# Autodesk Inventor assembly: DriveMotorAssem
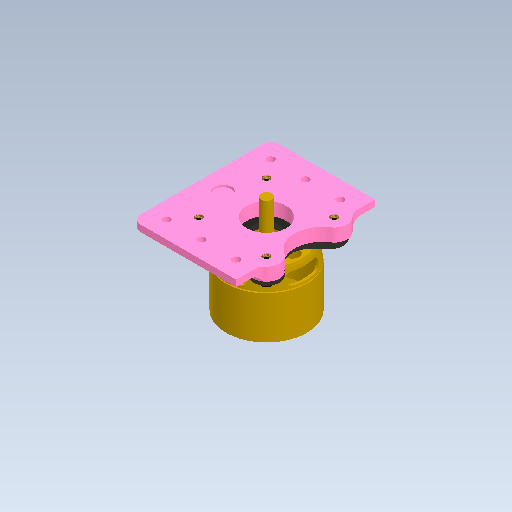
[picture p0: Inventor's stored thumbnail of the model, 512x512]
Saved by Autodesk Inventor 2023 (Build 270158000, 158)
## iProperties
Created: 2023-03-30
Part Number: DriveMotorAssem
Document SubType Name: Assembly
Designer: Dave
Mass: 268.152 g
Surface Area: 522.44 cm^2
Volume: 82.9291 cm^3
Density: 3.2335 g/cm^3
Author: Dave
## Documents named in this file (6)
- C:\Users\Dave\Documents\GitHub\BehrendURCMechanical\CAD\Chassis V3\DriveMotorAssem\DriveMotorAssem.iam
- C:\Users\Dave\Documents\GitHub\BehrendURCMechanical\CAD\Chassis V3\DriveMotorPlate.ipt
- C:\Users\Dave\Documents\GitHub\BehrendURCMechanical\CAD\Chassis V3\DriveMotorAssem\Drive Motor.ipt
- C:\Users\Dave\Downloads\91290A148_Alloy Steel Socket Head Screw.ipt
- C:\Users\Dave\Downloads\94180A351_Tapered Heat-Set Inserts for Plastic.ipt
- C:\Users\Dave\Documents\GitHub\BehrendURCMechanical\CAD\Chassis V3\DriveMotorAssem\DriveMotorMount4.ipt
## Components (11 placed, 5 different names)
1. DriveMotorMount4:2
2. DriveMotorPlate:1 — Insert:1, Insert:2, Insert:9, Insert:10, Insert:11, Insert:12
3. Drive Motor:1 — Insert:1, Insert:2
4. 91290A148_Alloy Steel Socket Head Screw:1 — Insert:9
5. 94180A351_Tapered Heat-Set Inserts for Plastic:1
6. 91290A148_Alloy Steel Socket Head Screw:2 — Insert:10
7. 94180A351_Tapered Heat-Set Inserts for Plastic:2
8. 91290A148_Alloy Steel Socket Head Screw:3 — Insert:11
9. 94180A351_Tapered Heat-Set Inserts for Plastic:3
10. 91290A148_Alloy Steel Socket Head Screw:4 — Insert:12
11. 94180A351_Tapered Heat-Set Inserts for Plastic:4
## Relationships (12: Insert 12)
- Insert:1: DriveMotorPlate:1 ↔ Drive Motor:1
- Insert:2: DriveMotorPlate:1 ↔ Drive Motor:1
- [Insert]: DriveMotorMount4:2 ↔ DriveMotorPlate:1
- [Insert]: DriveMotorMount4:2 ↔ DriveMotorPlate:1
- [Insert]: DriveMotorMount4:2 ↔ 94180A351_Tapered Heat-Set Inserts for Plastic:4
- [Insert]: DriveMotorMount4:2 ↔ 94180A351_Tapered Heat-Set Inserts for Plastic:1
- [Insert]: DriveMotorMount4:2 ↔ 94180A351_Tapered Heat-Set Inserts for Plastic:2
- [Insert]: DriveMotorMount4:2 ↔ 94180A351_Tapered Heat-Set Inserts for Plastic:3
- Insert:9: DriveMotorPlate:1 ↔ 91290A148_Alloy Steel Socket Head Screw:1
- Insert:10: DriveMotorPlate:1 ↔ 91290A148_Alloy Steel Socket Head Screw:2
- Insert:11: DriveMotorPlate:1 ↔ 91290A148_Alloy Steel Socket Head Screw:3
- Insert:12: DriveMotorPlate:1 ↔ 91290A148_Alloy Steel Socket Head Screw:4
